# Autodesk Inventor assembly: EFFECTOR
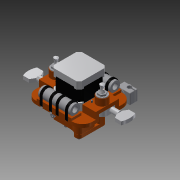
[picture p0: Inventor's stored thumbnail of the model, 180x180]
Saved by Autodesk Inventor 2013 (Build 170138000, 138)
## iProperties
Created: 2014-06-18
Part Number: EFFECTOR
Document SubType Name: Assembly
Designer: employee
Author: employee
## Documents named in this file (9)
- C:\Users\employee\Desktop\CoreXZ 2\EFFECTOR.iam
- C:\Users\employee\Desktop\CoreXZ 2\EFFECTOR PLATE.ipt
- C:\Users\employee\Desktop\CoreXZ 2\LM8UU.ipt
- C:\Users\employee\Desktop\CoreXZ 2\STEPPER.ipt
- C:\Users\employee\Desktop\CoreXZ 2\TUNING PEG.ipt
- C:\Users\employee\Desktop\CoreXZ 2\ZIP TIE EFFECTOR.ipt
- C:\Users\employee\Desktop\CoreXZ 2\TUNING PEG RETAINER.ipt
- C:\Users\employee\Desktop\CoreXZ 2\M2X10.ipt
- C:\Users\employee\Desktop\CoreXZ 2\EXTRUDER.iam
## Components (21 placed, 8 different names)
1. EFFECTOR PLATE:1 — Mate:1, Mate:2, Tangent:1, Tangent:2, Tangent:3, Tangent:4, Insert:3, Angle:1, Insert:5, Angle:2, Angle:3, Insert:6, Angle:4, Angle:5, Angle:6, Angle:7, Angle:8, Angle:9, Angle:10, Angle:11, Insert:15, Insert:16, Insert:19, Insert:20
2. LM8UU:1 — Insert:1, Mate:1, Insert:7, Insert:8
3. LM8UU:2 — Insert:1, Tangent:1, Tangent:2, Insert:9, Insert:10
4. LM8UU:3 — Insert:2, Tangent:3, Tangent:4, Insert:13, Insert:14
5. LM8UU:4 — Insert:2, Mate:2, Insert:11, Insert:12
6. STEPPER:1 — Insert:3, Angle:1
7. TUNING PEG:1 — Insert:5, Angle:3, Insert:18
8. TUNING PEG:2 — Angle:2, Insert:6, Insert:17
9. ZIP TIE EFFECTOR:1 — Insert:7, Angle:8
10. ZIP TIE EFFECTOR:2 — Insert:8, Angle:9
11. ZIP TIE EFFECTOR:3 — Insert:9, Angle:10
12. ZIP TIE EFFECTOR:4 — Insert:10, Angle:11
13. ZIP TIE EFFECTOR:5 — Insert:11, Angle:4
14. ZIP TIE EFFECTOR:6 — Insert:12, Angle:5
15. ZIP TIE EFFECTOR:7 — Insert:13, Angle:6
16. ZIP TIE EFFECTOR:8 — Insert:14, Angle:7
17. TUNING PEG RETAINER:1 — Insert:15
18. TUNING PEG RETAINER:2 — Insert:16
19. M2X10:1 — Insert:17
20. M2X10:2 — Insert:18
21. EXTRUDER:1 [sub-assembly] — Insert:19, Insert:20
## Relationships (36: Insert 19, Angle 11, Tangent 4, Mate 2)
- Insert:1: LM8UU:1 ↔ LM8UU:2
- Insert:2: LM8UU:3 ↔ LM8UU:4
- Mate:1: EFFECTOR PLATE:1 ↔ LM8UU:1
- Mate:2: EFFECTOR PLATE:1 ↔ LM8UU:4
- Tangent:1: EFFECTOR PLATE:1 ↔ LM8UU:2
- Tangent:2: EFFECTOR PLATE:1 ↔ LM8UU:2
- Tangent:3: EFFECTOR PLATE:1 ↔ LM8UU:3
- Tangent:4: EFFECTOR PLATE:1 ↔ LM8UU:3
- Insert:3: EFFECTOR PLATE:1 ↔ STEPPER:1
- Angle:1 (0 deg): EFFECTOR PLATE:1 ↔ STEPPER:1
- Insert:5: EFFECTOR PLATE:1 ↔ TUNING PEG:1
- Angle:2 (0 deg): EFFECTOR PLATE:1 ↔ TUNING PEG:2
- Angle:3 (0 deg): EFFECTOR PLATE:1 ↔ TUNING PEG:1
- Insert:6: EFFECTOR PLATE:1 ↔ TUNING PEG:2
- Insert:7 (3.25 mm): LM8UU:1 ↔ ZIP TIE EFFECTOR:1
- Insert:8 (3.25 mm): LM8UU:1 ↔ ZIP TIE EFFECTOR:2
- Insert:9 (3.25 mm): LM8UU:2 ↔ ZIP TIE EFFECTOR:3
- Insert:10 (3.25 mm): LM8UU:2 ↔ ZIP TIE EFFECTOR:4
- Insert:11 (3.25 mm): LM8UU:4 ↔ ZIP TIE EFFECTOR:5
- Insert:12 (3.25 mm): LM8UU:4 ↔ ZIP TIE EFFECTOR:6
- Insert:13 (3.25 mm): LM8UU:3 ↔ ZIP TIE EFFECTOR:7
- Insert:14 (3.25 mm): LM8UU:3 ↔ ZIP TIE EFFECTOR:8
- Angle:4 (0 deg): EFFECTOR PLATE:1 ↔ ZIP TIE EFFECTOR:5
- Angle:5 (0 deg): EFFECTOR PLATE:1 ↔ ZIP TIE EFFECTOR:6
- Angle:6 (0 deg): EFFECTOR PLATE:1 ↔ ZIP TIE EFFECTOR:7
- Angle:7 (0 deg): EFFECTOR PLATE:1 ↔ ZIP TIE EFFECTOR:8
- Angle:8 (0 deg): EFFECTOR PLATE:1 ↔ ZIP TIE EFFECTOR:1
- Angle:9 (0 deg): EFFECTOR PLATE:1 ↔ ZIP TIE EFFECTOR:2
- Angle:10 (0 deg): EFFECTOR PLATE:1 ↔ ZIP TIE EFFECTOR:3
- Angle:11 (0 deg): EFFECTOR PLATE:1 ↔ ZIP TIE EFFECTOR:4
- Insert:15: EFFECTOR PLATE:1 ↔ TUNING PEG RETAINER:1
- Insert:16: EFFECTOR PLATE:1 ↔ TUNING PEG RETAINER:2
- Insert:17: TUNING PEG:2 ↔ M2X10:1
- Insert:18: TUNING PEG:1 ↔ M2X10:2
- Insert:19: EFFECTOR PLATE:1 ↔ EXTRUDER:1
- Insert:20: EFFECTOR PLATE:1 ↔ EXTRUDER:1
